# Autodesk Inventor assembly: rotBaseCase
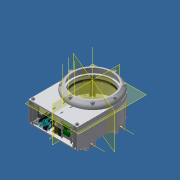
[picture p0: Inventor's stored thumbnail of the model, 180x180]
Saved by Autodesk Inventor 2016 (Build 200138000, 138)
## iProperties
Created: 2016-02-29
Part Number: rotBaseCase
Material: Generisch
Document SubType Name: Assembly
Designer: 4ndreas
Mass: 3728.71 g
Surface Area: 10018.9 cm^2
Volume: 2081.83 cm^3
Density: 1.79108 g/cm^3
Parent: World
Author: 4ndreas
## Documents named in this file (20)
- C:\Users\4ndreas\Documents\github\Mantis-Robot-Arm\MantisRobotArm\Workspace\_assemblys\rotBaseCase.iam
- C:\Users\4ndreas\Documents\github\Mantis-Robot-Arm\MantisRobotArm\Workspace\_metal parts\BasePlate_B.ipt
- C:\Users\4ndreas\Documents\github\Mantis-Robot-Arm\MantisRobotArm\Workspace\_printed parts\BaseBearingMount.ipt
- C:\Users\4ndreas\Documents\github\Mantis-Robot-Arm\MantisRobotArm\Workspace\_assemblys\RotMotor.iam
- C:\Users\4ndreas\Documents\github\Mantis-Robot-Arm\MantisRobotArm\Workspace\_metal parts\Alu_Cover_A.ipt
- C:\Users\4ndreas\Documents\github\Mantis-Robot-Arm\MantisRobotArm\Workspace\_standard Parts\GummiFeet.ipt
- C:\Users\4ndreas\Documents\github\Mantis-Robot-Arm\MantisRobotArm\Libraries\Content Center Files\de-DE\DIN 912\DIN 912 - M5 x 0,8 x 16 x 14.ipt
- C:\Users\4ndreas\Documents\github\Mantis-Robot-Arm\MantisRobotArm\Libraries\Content Center Files\de-DE\DIN 9021\DIN 9021 - 5,3.ipt
- C:\Users\4ndreas\Documents\github\Mantis-Robot-Arm\MantisRobotArm\Workspace\_motors\StepperDriver.ipt
- C:\Users\4ndreas\Documents\github\Mantis-Robot-Arm\MantisRobotArm\Workspace\_metal parts\CAP 0_0_370_03_000   Profil 5  20x20 natur-.ipt
- C:\Users\4ndreas\Documents\github\Mantis-Robot-Arm\MantisRobotArm\Workspace\_metal parts\DriverMount.ipt
- C:\Users\4ndreas\Documents\github\Mantis-Robot-Arm\MantisRobotArm\Libraries\Content Center Files\de-DE\ISO 7380-1\ISO 7380-1 - M3 x 6.ipt
- C:\Users\4ndreas\Documents\github\Mantis-Robot-Arm\MantisRobotArm\Libraries\Content Center Files\de-DE\DIN 912\DIN 912 - M4 x 0,7 x 40 x 20.ipt
- C:\Users\4ndreas\Documents\github\Mantis-Robot-Arm\MantisRobotArm\Libraries\Content Center Files\de-DE\DIN 912\DIN 912 - M4 x 0,7 x 25 x 23,25.ipt
- C:\Users\4ndreas\Documents\github\Mantis-Robot-Arm\MantisRobotArm\Workspace\_metal parts\Distanzhuelse_M3x5mm_.ipt
- C:\Users\4ndreas\Documents\github\Mantis-Robot-Arm\MantisRobotArm\Workspace\_metal parts\Distanzhuelse_M3x20mm_.ipt
- C:\Users\4ndreas\Documents\github\Mantis-Robot-Arm\MantisRobotArm\Workspace\_metal parts\BasePlate_base.ipt
- C:\Users\4ndreas\Documents\github\Mantis-Robot-Arm\MantisRobotArm\Libraries\Content Center Files\arduino due.ipt
- C:\Users\4ndreas\Documents\github\Mantis-Robot-Arm\MantisRobotArm\Workspace\_printed parts\_baseBearingMount.ipt
- C:\Users\4ndreas\Documents\github\Mantis-Robot-Arm\MantisRobotArm\Workspace\_standard Parts\Linearwagen_16_kurz.ipt
## Components (86 placed, 19 different names)
1. BasePlate_base:1 — Passend:2, Passend:11, Passend:12, Passend:13, Passend:14, Passend:15, Passend:16, Passend:17, Passend:18, Passend:19, Passend:20, Passend:21, Passend:22, Passend:34, Fluchtend:8, Passend:36, Passend:37, Passend:40, Passend:41, Passend:42, Passend:119, Passend:163, Passend:172, Passend:173, Fluchtend:42, Passend:183, Passend:184, Tangential:2, Winkel:1, Tangential:3, Passend:187, Passend:188
2. BasePlate_B:1 — Passend:1, Passend:2, Passend:3, Passend:4, Passend:5, Passend:6, Passend:10, Fluchtend:4, Passend:25, Passend:28, Passend:29, Passend:30, Passend:35, Passend:38, Passend:39, Fluchtend:9, Passend:43, Passend:44, Passend:45, Fluchtend:10, Fluchtend:11, Passend:182, Winkel:2
3. BaseBearingMount:1 — Passend:4, Passend:5, Passend:108, Einfügen:1, Einfügen:2, Einfügen:3, Einfügen:4, Einfügen:5, Einfügen:6, Einfügen:7, Einfügen:8
4. RotMotor:1 [sub-assembly] — Passend:6, Passend:9, Passend:1, Passend:182, Passend:190
5. Alu_Cover_A:1 — Passend:9, Passend:10, Fluchtend:4, Tangential:1
6. GummiFeet:1 — Passend:11, Passend:12
7. GummiFeet:2 — Passend:13, Passend:20
8. GummiFeet:3 — Passend:15, Passend:18, Passend:3
9. GummiFeet:4 — Passend:14, Passend:19
10. GummiFeet:5 — Passend:17, Passend:21
11. GummiFeet:6 — Passend:16, Passend:22
12. DIN 912 - ersetzt durch DIN EN ISO 4762 M5 x 16:1 — Passend:23, Passend:24, Passend:25
13. DIN 9021 5,3:1 — Passend:23, Passend:24, Passend:28
14. DIN 912 - ersetzt durch DIN EN ISO 4762 M5 x 16:2 — Passend:29
15. DIN 9021 5,3:2 — Passend:30
16. CAP 0_0_370_03_000   Profil 5  20x20 natur-:1 — Passend:34, Passend:35, Fluchtend:8, Fluchtend:32, Passend:61, Passend:63, Passend:72, Fluchtend:37
17. CAP 0_0_370_03_000   Profil 5  20x20 natur-:2 — Passend:36, Passend:38, Fluchtend:9, Passend:62, Fluchtend:40
18. CAP 0_0_370_03_000   Profil 5  20x20 natur-:3 — Passend:37, Passend:39, Passend:108
19. CAP 0_0_370_03_000   Profil 5  20x20 natur-:4 — Passend:40, Passend:44
20. CAP 0_0_370_03_000   Profil 5  20x20 natur-:5 — Passend:41, Passend:45, Fluchtend:10, Fluchtend:35, Passend:66, Passend:67, Fluchtend:41, Passend:180
21. CAP 0_0_370_03_000   Profil 5  20x20 natur-:6 — Passend:42, Passend:43, Fluchtend:11
22. StepperDriver:6 — Fluchtend:23, Fluchtend:24, Passend:62, Passend:64, Passend:74, Passend:75, Passend:76, Passend:77, Passend:78, Passend:79, Passend:80, Passend:81
23. StepperDriver:8 — Fluchtend:23, Fluchtend:24, Fluchtend:32, Fluchtend:34, Passend:61, Passend:65, Passend:82, Passend:83, Passend:84, Passend:85, Passend:86, Passend:87, Passend:88, Passend:89, Passend:90, Passend:91
24. StepperDriver:10 — Fluchtend:33, Fluchtend:35, Fluchtend:36, Passend:70, Passend:71, Passend:100, Passend:101, Passend:102, Passend:103, Passend:104, Passend:105, Passend:106, Passend:107
25. StepperDriver:11 — Fluchtend:33, Fluchtend:34, Fluchtend:36, Passend:68, Passend:69, Passend:92, Passend:93, Passend:94, Passend:95, Passend:96, Passend:97, Passend:98, Passend:99
26. StepperDriver:12 — Fluchtend:37, Fluchtend:38, Fluchtend:39, Passend:72, Passend:117, Passend:118, Passend:120, Passend:121, Passend:122, Passend:123, Passend:124, Passend:125, Passend:126, Passend:127, Passend:140, Passend:141, Passend:142
27. StepperDriver:13 — Fluchtend:38, Fluchtend:39, Passend:130, Passend:137, Passend:138, Passend:139, Passend:143, Passend:144, Passend:145, Passend:146, Passend:147, Passend:148, Passend:149, Passend:150
28. DriverMount:1 — Fluchtend:40
29. DriverMount:2 — Passend:63, Passend:64, Passend:65
30. DriverMount:3 — Passend:67, Passend:69, Passend:71
31. DriverMount:4 — Passend:66, Passend:68, Passend:70, Fluchtend:41
32. ISO 7380-1 M3 x 6:1 — Passend:74, Passend:75
33. ISO 7380-1 M3 x 6:2 — Passend:76, Passend:77
34. ISO 7380-1 M3 x 6:3 — Passend:78, Passend:79
35. ISO 7380-1 M3 x 6:4 — Passend:80, Passend:81
36. ISO 7380-1 M3 x 6:5 — Passend:82, Passend:83
37. ISO 7380-1 M3 x 6:6 — Passend:84, Passend:85
38. ISO 7380-1 M3 x 6:7 — Passend:86, Passend:87
39. ISO 7380-1 M3 x 6:8 — Passend:88, Passend:89
40. ISO 7380-1 M3 x 6:9 — Passend:90, Passend:91
41. ISO 7380-1 M3 x 6:10 — Passend:92, Passend:93
42. ISO 7380-1 M3 x 6:11 — Passend:94, Passend:95
43. ISO 7380-1 M3 x 6:12 — Passend:96, Passend:97
44. ISO 7380-1 M3 x 6:13 — Passend:98, Passend:99
45. ISO 7380-1 M3 x 6:14 — Passend:100, Passend:101
46. ISO 7380-1 M3 x 6:15 — Passend:102, Passend:103
47. ISO 7380-1 M3 x 6:16 — Passend:104, Passend:105
48. ISO 7380-1 M3 x 6:17 — Passend:106, Passend:107
49. DIN 912 - ersetzt durch DIN EN ISO 4762 M4 x 40:1 — Einfügen:1
50. DIN 912 - ersetzt durch DIN EN ISO 4762 M4 x 25:2 — Einfügen:2
51. DIN 912 - ersetzt durch DIN EN ISO 4762 M4 x 25:5 — Einfügen:3
52. DIN 912 - ersetzt durch DIN EN ISO 4762 M4 x 25:6 — Einfügen:4
53. DIN 912 - ersetzt durch DIN EN ISO 4762 M4 x 25:4 — Einfügen:5
54. DIN 912 - ersetzt durch DIN EN ISO 4762 M4 x 25:3 — Einfügen:6
55. DIN 912 - ersetzt durch DIN EN ISO 4762 M4 x 40:7 — Einfügen:7
56. DIN 912 - ersetzt durch DIN EN ISO 4762 M4 x 25:1 — Einfügen:8
57. Distanzhuelse_M3x5mm_:1 — Passend:163, Passend:164, Passend:166
58. Distanzhuelse_M3x20mm_:1 — Passend:117, Passend:118, Passend:119
59. Distanzhuelse_M3x5mm_:3 — Passend:174, Passend:177
60. Distanzhuelse_M3x5mm_:4 — Passend:175, Passend:176
61. Distanzhuelse_M3x5mm_:5 — Passend:178, Passend:179
62. Distanzhuelse_M3x20mm_:2 — Passend:122, Passend:123
63. Distanzhuelse_M3x20mm_:3 — Passend:121, Passend:124
64. Distanzhuelse_M3x20mm_:4 — Passend:120, Passend:125
65. Distanzhuelse_M3x20mm_:5 — Passend:126, Passend:127, Passend:128, Passend:129
66. Distanzhuelse_M3x20mm_:6 — Passend:128, Passend:129, Passend:130
67. Distanzhuelse_M3x20mm_:7 — Passend:131, Passend:134, Passend:142
68. Distanzhuelse_M3x20mm_:8 — Passend:132, Passend:135, Passend:140
69. Distanzhuelse_M3x20mm_:9 — Passend:131, Passend:134, Passend:137
70. Distanzhuelse_M3x20mm_:10 — Passend:132, Passend:135, Passend:138
71. Distanzhuelse_M3x20mm_:11 — Passend:133, Passend:136, Passend:141
72. Distanzhuelse_M3x20mm_:12 — Passend:133, Passend:136, Passend:139
73. ISO 7380-1 M3 x 6:18 — Passend:143, Passend:144
74. ISO 7380-1 M3 x 6:19 — Passend:145, Passend:146
75. ISO 7380-1 M3 x 6:20 — Passend:147, Passend:148
76. ISO 7380-1 M3 x 6:21 — Passend:149, Passend:150
77. ISO 7380-1 M3 x 6:22 — Passend:165, Passend:166
78. ISO 7380-1 M3 x 6:25 — Passend:168, Passend:169, Passend:174
79. ISO 7380-1 M3 x 6:26 — Passend:170, Passend:171, Passend:175
80. ISO 7380-1 M3 x 6:27 — Passend:167, Passend:178
81. arduino due:1 — Passend:164, Passend:165, Passend:167, Passend:168, Passend:169, Passend:170, Passend:171, Passend:176, Passend:177, Fluchtend:42, Passend:179, Passend:180
82. _baseBearingMount:1 — Passend:172, Passend:173, Passend:191
83. Linearwagen_16_kurz:1 — Passend:183, Passend:185, Tangential:1, Tangential:2, Winkel:1, Fluchtend:43
84. Linearwagen_16_kurz:2 — Passend:184, Passend:185, Tangential:3, Fluchtend:44, Passend:189
85. Linearwagen_16_kurz:3 — Passend:186, Passend:187, Fluchtend:43
86. Linearwagen_16_kurz:4 — Passend:186, Passend:188, Fluchtend:44, Passend:189
## Relationships (185: Mate 149, Flush 23, Insert 8, Tangent 3, Angle 2)
- Passend:1 [Mate]: BasePlate_B:1 ↔ RotMotor:1
- Passend:2 [Mate] (85 mm): BasePlate_base:1 ↔ BasePlate_B:1
- Passend:3 [Mate]: BasePlate_B:1 ↔ GummiFeet:3
- [Flush]: BasePlate_base:1
- [Flush]: BasePlate_base:1
- [Flush]: BasePlate_base:1
- Passend:4 [Mate]: BasePlate_B:1 ↔ BaseBearingMount:1
- Passend:5 [Mate]: BasePlate_B:1 ↔ BaseBearingMount:1
- Passend:6 [Mate]: BasePlate_B:1 ↔ RotMotor:1
- Passend:9 [Mate]: RotMotor:1 ↔ Alu_Cover_A:1
- Passend:10 [Mate]: BasePlate_B:1 ↔ Alu_Cover_A:1
- Fluchtend:4 [Flush]: BasePlate_B:1 ↔ Alu_Cover_A:1
- Passend:11 [Mate]: BasePlate_base:1 ↔ GummiFeet:1
- Passend:12 [Mate]: BasePlate_base:1 ↔ GummiFeet:1
- Passend:13 [Mate]: BasePlate_base:1 ↔ GummiFeet:2
- Passend:14 [Mate]: BasePlate_base:1 ↔ GummiFeet:4
- Passend:15 [Mate]: BasePlate_base:1 ↔ GummiFeet:3
- Passend:16 [Mate]: BasePlate_base:1 ↔ GummiFeet:6
- Passend:17 [Mate]: BasePlate_base:1 ↔ GummiFeet:5
- Passend:18 [Mate]: BasePlate_base:1 ↔ GummiFeet:3
- Passend:19 [Mate]: BasePlate_base:1 ↔ GummiFeet:4
- Passend:20 [Mate]: BasePlate_base:1 ↔ GummiFeet:2
- Passend:21 [Mate]: BasePlate_base:1 ↔ GummiFeet:5
- Passend:22 [Mate]: BasePlate_base:1 ↔ GummiFeet:6
- Passend:23 [Mate]: DIN 912 - ersetzt durch DIN EN ISO 4762 M5 x 16:1 ↔ DIN 9021 5,3:1
- Passend:24 [Mate]: DIN 912 - ersetzt durch DIN EN ISO 4762 M5 x 16:1 ↔ DIN 9021 5,3:1
- Passend:25 [Mate]: BasePlate_B:1 ↔ DIN 912 - ersetzt durch DIN EN ISO 4762 M5 x 16:1
- [Mate]: DIN 912 - ersetzt durch DIN EN ISO 4762 M5 x 16:2 ↔ DIN 9021 5,3:2
- [Mate]: DIN 912 - ersetzt durch DIN EN ISO 4762 M5 x 16:2 ↔ DIN 9021 5,3:2
- Passend:28 [Mate]: BasePlate_B:1 ↔ DIN 9021 5,3:1
- Passend:29 [Mate]: BasePlate_B:1 ↔ DIN 912 - ersetzt durch DIN EN ISO 4762 M5 x 16:2
- Passend:30 [Mate]: BasePlate_B:1 ↔ DIN 9021 5,3:2
- Passend:34 [Mate]: BasePlate_base:1 ↔ CAP 0_0_370_03_000   Profil 5  20x20 natur-:1
- Passend:35 [Mate]: BasePlate_B:1 ↔ CAP 0_0_370_03_000   Profil 5  20x20 natur-:1
- Fluchtend:8 [Flush]: BasePlate_base:1 ↔ CAP 0_0_370_03_000   Profil 5  20x20 natur-:1
- Passend:36 [Mate]: BasePlate_base:1 ↔ CAP 0_0_370_03_000   Profil 5  20x20 natur-:2
- Passend:37 [Mate]: BasePlate_base:1 ↔ CAP 0_0_370_03_000   Profil 5  20x20 natur-:3
- Passend:38 [Mate]: BasePlate_B:1 ↔ CAP 0_0_370_03_000   Profil 5  20x20 natur-:2
- Passend:39 [Mate]: BasePlate_B:1 ↔ CAP 0_0_370_03_000   Profil 5  20x20 natur-:3
- Fluchtend:9 [Flush]: BasePlate_B:1 ↔ CAP 0_0_370_03_000   Profil 5  20x20 natur-:2
- Passend:40 [Mate]: BasePlate_base:1 ↔ CAP 0_0_370_03_000   Profil 5  20x20 natur-:4
- Passend:41 [Mate]: BasePlate_base:1 ↔ CAP 0_0_370_03_000   Profil 5  20x20 natur-:5
- Passend:42 [Mate]: BasePlate_base:1 ↔ CAP 0_0_370_03_000   Profil 5  20x20 natur-:6
- Passend:43 [Mate]: BasePlate_B:1 ↔ CAP 0_0_370_03_000   Profil 5  20x20 natur-:6
- Passend:44 [Mate]: BasePlate_B:1 ↔ CAP 0_0_370_03_000   Profil 5  20x20 natur-:4
- Passend:45 [Mate]: BasePlate_B:1 ↔ CAP 0_0_370_03_000   Profil 5  20x20 natur-:5
- Fluchtend:10 [Flush]: BasePlate_B:1 ↔ CAP 0_0_370_03_000   Profil 5  20x20 natur-:5
- Fluchtend:11 [Flush]: BasePlate_B:1 ↔ CAP 0_0_370_03_000   Profil 5  20x20 natur-:6
- Fluchtend:23 [Flush]: StepperDriver:6 ↔ StepperDriver:8
- Fluchtend:24 [Flush]: StepperDriver:6 ↔ StepperDriver:8
- Fluchtend:32 [Flush]: CAP 0_0_370_03_000   Profil 5  20x20 natur-:1 ↔ StepperDriver:8
- Fluchtend:33 [Flush]: StepperDriver:10 ↔ StepperDriver:11
- Fluchtend:34 [Flush]: StepperDriver:8 ↔ StepperDriver:11
- Fluchtend:35 [Flush]: CAP 0_0_370_03_000   Profil 5  20x20 natur-:5 ↔ StepperDriver:10
- Fluchtend:36 [Flush]: StepperDriver:10 ↔ StepperDriver:11
- Fluchtend:37 [Flush] (10 mm): CAP 0_0_370_03_000   Profil 5  20x20 natur-:1 ↔ StepperDriver:12
- Fluchtend:38 [Flush]: StepperDriver:12 ↔ StepperDriver:13
- Fluchtend:39 [Flush]: StepperDriver:12 ↔ StepperDriver:13
- Passend:61 [Mate] (2 mm): CAP 0_0_370_03_000   Profil 5  20x20 natur-:1 ↔ StepperDriver:8
- Passend:62 [Mate] (2 mm): CAP 0_0_370_03_000   Profil 5  20x20 natur-:2 ↔ StepperDriver:6
- Fluchtend:40 [Flush]: CAP 0_0_370_03_000   Profil 5  20x20 natur-:2 ↔ DriverMount:1
- Passend:63 [Mate]: CAP 0_0_370_03_000   Profil 5  20x20 natur-:1 ↔ DriverMount:2
- Passend:64 [Mate]: StepperDriver:6 ↔ DriverMount:2
- Passend:65 [Mate]: StepperDriver:8 ↔ DriverMount:2
- Passend:66 [Mate]: CAP 0_0_370_03_000   Profil 5  20x20 natur-:5 ↔ DriverMount:4
- Passend:67 [Mate]: CAP 0_0_370_03_000   Profil 5  20x20 natur-:5 ↔ DriverMount:3
- Passend:68 [Mate]: StepperDriver:11 ↔ DriverMount:4
- Passend:69 [Mate]: StepperDriver:11 ↔ DriverMount:3
- Passend:70 [Mate]: StepperDriver:10 ↔ DriverMount:4
- Fluchtend:41 [Flush]: CAP 0_0_370_03_000   Profil 5  20x20 natur-:5 ↔ DriverMount:4
- Passend:71 [Mate]: StepperDriver:10 ↔ DriverMount:3
- Passend:72 [Mate] (16 mm): CAP 0_0_370_03_000   Profil 5  20x20 natur-:1 ↔ StepperDriver:12
- Passend:74 [Mate]: StepperDriver:6 ↔ ISO 7380-1 M3 x 6:1
- Passend:75 [Mate]: StepperDriver:6 ↔ ISO 7380-1 M3 x 6:1
- Passend:76 [Mate]: StepperDriver:6 ↔ ISO 7380-1 M3 x 6:2
- Passend:77 [Mate]: StepperDriver:6 ↔ ISO 7380-1 M3 x 6:2
- Passend:78 [Mate]: StepperDriver:6 ↔ ISO 7380-1 M3 x 6:3
- Passend:79 [Mate]: StepperDriver:6 ↔ ISO 7380-1 M3 x 6:3
- Passend:80 [Mate]: StepperDriver:6 ↔ ISO 7380-1 M3 x 6:4
- Passend:81 [Mate]: StepperDriver:6 ↔ ISO 7380-1 M3 x 6:4
- Passend:82 [Mate]: StepperDriver:8 ↔ ISO 7380-1 M3 x 6:5
- Passend:83 [Mate]: StepperDriver:8 ↔ ISO 7380-1 M3 x 6:5
- Passend:84 [Mate]: StepperDriver:8 ↔ ISO 7380-1 M3 x 6:6
- Passend:85 [Mate]: StepperDriver:8 ↔ ISO 7380-1 M3 x 6:6
- Passend:86 [Mate]: StepperDriver:8 ↔ ISO 7380-1 M3 x 6:7
- Passend:87 [Mate]: StepperDriver:8 ↔ ISO 7380-1 M3 x 6:7
- Passend:88 [Mate]: StepperDriver:8 ↔ ISO 7380-1 M3 x 6:8
- Passend:89 [Mate]: StepperDriver:8 ↔ ISO 7380-1 M3 x 6:8
- Passend:90 [Mate]: StepperDriver:8 ↔ ISO 7380-1 M3 x 6:9
- Passend:91 [Mate]: StepperDriver:8 ↔ ISO 7380-1 M3 x 6:9
- Passend:92 [Mate]: StepperDriver:11 ↔ ISO 7380-1 M3 x 6:10
- Passend:93 [Mate]: StepperDriver:11 ↔ ISO 7380-1 M3 x 6:10
- Passend:94 [Mate]: StepperDriver:11 ↔ ISO 7380-1 M3 x 6:11
- Passend:95 [Mate]: StepperDriver:11 ↔ ISO 7380-1 M3 x 6:11
- Passend:96 [Mate]: StepperDriver:11 ↔ ISO 7380-1 M3 x 6:12
- Passend:97 [Mate]: StepperDriver:11 ↔ ISO 7380-1 M3 x 6:12
- Passend:98 [Mate]: StepperDriver:11 ↔ ISO 7380-1 M3 x 6:13
- Passend:99 [Mate]: StepperDriver:11 ↔ ISO 7380-1 M3 x 6:13
- Passend:100 [Mate]: StepperDriver:10 ↔ ISO 7380-1 M3 x 6:14
- Passend:101 [Mate]: StepperDriver:10 ↔ ISO 7380-1 M3 x 6:14
- Passend:102 [Mate]: StepperDriver:10 ↔ ISO 7380-1 M3 x 6:15
- Passend:103 [Mate]: StepperDriver:10 ↔ ISO 7380-1 M3 x 6:15
- Passend:104 [Mate]: StepperDriver:10 ↔ ISO 7380-1 M3 x 6:16
- Passend:105 [Mate]: StepperDriver:10 ↔ ISO 7380-1 M3 x 6:16
- Passend:106 [Mate]: StepperDriver:10 ↔ ISO 7380-1 M3 x 6:17
- Passend:107 [Mate]: StepperDriver:10 ↔ ISO 7380-1 M3 x 6:17
- Passend:108 [Mate]: BaseBearingMount:1 ↔ CAP 0_0_370_03_000   Profil 5  20x20 natur-:3
- Einfügen:1 [Insert]: BaseBearingMount:1 ↔ DIN 912 - ersetzt durch DIN EN ISO 4762 M4 x 40:1
- Einfügen:2 [Insert]: BaseBearingMount:1 ↔ DIN 912 - ersetzt durch DIN EN ISO 4762 M4 x 25:2
- Einfügen:3 [Insert]: BaseBearingMount:1 ↔ DIN 912 - ersetzt durch DIN EN ISO 4762 M4 x 25:5
- Einfügen:4 [Insert]: BaseBearingMount:1 ↔ DIN 912 - ersetzt durch DIN EN ISO 4762 M4 x 25:6
- Einfügen:5 [Insert]: BaseBearingMount:1 ↔ DIN 912 - ersetzt durch DIN EN ISO 4762 M4 x 25:4
- Einfügen:6 [Insert]: BaseBearingMount:1 ↔ DIN 912 - ersetzt durch DIN EN ISO 4762 M4 x 25:3
- Einfügen:7 [Insert]: BaseBearingMount:1 ↔ DIN 912 - ersetzt durch DIN EN ISO 4762 M4 x 40:7
- Einfügen:8 [Insert]: BaseBearingMount:1 ↔ DIN 912 - ersetzt durch DIN EN ISO 4762 M4 x 25:1
- Passend:117 [Mate]: StepperDriver:12 ↔ Distanzhuelse_M3x20mm_:1
- Passend:118 [Mate]: StepperDriver:12 ↔ Distanzhuelse_M3x20mm_:1
- Passend:119 [Mate]: BasePlate_base:1 ↔ Distanzhuelse_M3x20mm_:1
- Passend:120 [Mate]: StepperDriver:12 ↔ Distanzhuelse_M3x20mm_:4
- Passend:121 [Mate]: StepperDriver:12 ↔ Distanzhuelse_M3x20mm_:3
- Passend:122 [Mate]: StepperDriver:12 ↔ Distanzhuelse_M3x20mm_:2
- Passend:123 [Mate]: StepperDriver:12 ↔ Distanzhuelse_M3x20mm_:2
- Passend:124 [Mate]: StepperDriver:12 ↔ Distanzhuelse_M3x20mm_:3
- Passend:125 [Mate]: StepperDriver:12 ↔ Distanzhuelse_M3x20mm_:4
- Passend:126 [Mate]: StepperDriver:12 ↔ Distanzhuelse_M3x20mm_:5
- Passend:127 [Mate]: StepperDriver:12 ↔ Distanzhuelse_M3x20mm_:5
- Passend:128 [Mate]: Distanzhuelse_M3x20mm_:5 ↔ Distanzhuelse_M3x20mm_:6
- Passend:129 [Mate]: Distanzhuelse_M3x20mm_:5 ↔ Distanzhuelse_M3x20mm_:6
- Passend:130 [Mate]: StepperDriver:13 ↔ Distanzhuelse_M3x20mm_:6
- Passend:131 [Mate]: Distanzhuelse_M3x20mm_:7 ↔ Distanzhuelse_M3x20mm_:9
- Passend:132 [Mate]: Distanzhuelse_M3x20mm_:8 ↔ Distanzhuelse_M3x20mm_:10
- Passend:133 [Mate]: Distanzhuelse_M3x20mm_:11 ↔ Distanzhuelse_M3x20mm_:12
- Passend:134 [Mate]: Distanzhuelse_M3x20mm_:7 ↔ Distanzhuelse_M3x20mm_:9
- Passend:135 [Mate]: Distanzhuelse_M3x20mm_:8 ↔ Distanzhuelse_M3x20mm_:10
- Passend:136 [Mate]: Distanzhuelse_M3x20mm_:11 ↔ Distanzhuelse_M3x20mm_:12
- Passend:137 [Mate]: StepperDriver:13 ↔ Distanzhuelse_M3x20mm_:9
- Passend:138 [Mate]: StepperDriver:13 ↔ Distanzhuelse_M3x20mm_:10
- Passend:139 [Mate]: StepperDriver:13 ↔ Distanzhuelse_M3x20mm_:12
- Passend:140 [Mate]: StepperDriver:12 ↔ Distanzhuelse_M3x20mm_:8
- Passend:141 [Mate]: StepperDriver:12 ↔ Distanzhuelse_M3x20mm_:11
- Passend:142 [Mate]: StepperDriver:12 ↔ Distanzhuelse_M3x20mm_:7
- Passend:143 [Mate]: StepperDriver:13 ↔ ISO 7380-1 M3 x 6:18
- Passend:144 [Mate]: StepperDriver:13 ↔ ISO 7380-1 M3 x 6:18
- Passend:145 [Mate]: StepperDriver:13 ↔ ISO 7380-1 M3 x 6:19
- Passend:146 [Mate]: StepperDriver:13 ↔ ISO 7380-1 M3 x 6:19
- Passend:147 [Mate]: StepperDriver:13 ↔ ISO 7380-1 M3 x 6:20
- Passend:148 [Mate]: StepperDriver:13 ↔ ISO 7380-1 M3 x 6:20
- Passend:149 [Mate]: StepperDriver:13 ↔ ISO 7380-1 M3 x 6:21
- Passend:150 [Mate]: StepperDriver:13 ↔ ISO 7380-1 M3 x 6:21
- Passend:163 [Mate]: BasePlate_base:1 ↔ Distanzhuelse_M3x5mm_:1
- Passend:164 [Mate]: Distanzhuelse_M3x5mm_:1 ↔ arduino due:1
- Passend:165 [Mate]: ISO 7380-1 M3 x 6:22 ↔ arduino due:1
- Passend:166 [Mate]: Distanzhuelse_M3x5mm_:1 ↔ ISO 7380-1 M3 x 6:22
- Passend:167 [Mate]: ISO 7380-1 M3 x 6:27 ↔ arduino due:1
- Passend:168 [Mate]: ISO 7380-1 M3 x 6:25 ↔ arduino due:1
- Passend:169 [Mate]: ISO 7380-1 M3 x 6:25 ↔ arduino due:1
- Passend:170 [Mate]: ISO 7380-1 M3 x 6:26 ↔ arduino due:1
- Passend:171 [Mate]: ISO 7380-1 M3 x 6:26 ↔ arduino due:1
- Passend:172 [Mate]: BasePlate_base:1 ↔ _baseBearingMount:1
- Passend:173 [Mate]: BasePlate_base:1 ↔ _baseBearingMount:1
- Passend:174 [Mate]: Distanzhuelse_M3x5mm_:3 ↔ ISO 7380-1 M3 x 6:25
- Passend:175 [Mate]: Distanzhuelse_M3x5mm_:4 ↔ ISO 7380-1 M3 x 6:26
- Passend:176 [Mate]: Distanzhuelse_M3x5mm_:4 ↔ arduino due:1
- Passend:177 [Mate]: Distanzhuelse_M3x5mm_:3 ↔ arduino due:1
- Fluchtend:42 [Flush]: BasePlate_base:1 ↔ arduino due:1
- Passend:178 [Mate]: Distanzhuelse_M3x5mm_:5 ↔ ISO 7380-1 M3 x 6:27
- Passend:179 [Mate]: Distanzhuelse_M3x5mm_:5 ↔ arduino due:1
- Passend:180 [Mate] (8 mm): CAP 0_0_370_03_000   Profil 5  20x20 natur-:5 ↔ arduino due:1
- Passend:182 [Mate]: BasePlate_B:1 ↔ RotMotor:1
- Passend:183 [Mate]: BasePlate_base:1 ↔ Linearwagen_16_kurz:1
- Passend:184 [Mate]: BasePlate_base:1 ↔ Linearwagen_16_kurz:2
- Passend:185 [Mate]: Linearwagen_16_kurz:1 ↔ Linearwagen_16_kurz:2
- Tangential:1: Alu_Cover_A:1 ↔ Linearwagen_16_kurz:1
- Tangential:2: BasePlate_base:1 ↔ Linearwagen_16_kurz:1
- Winkel:1 [Angle] (0 deg): BasePlate_base:1 ↔ Linearwagen_16_kurz:1
- Tangential:3: BasePlate_base:1 ↔ Linearwagen_16_kurz:2
- Passend:186 [Mate]: Linearwagen_16_kurz:3 ↔ Linearwagen_16_kurz:4
- Passend:187 [Mate]: BasePlate_base:1 ↔ Linearwagen_16_kurz:3
- Passend:188 [Mate]: BasePlate_base:1 ↔ Linearwagen_16_kurz:4
- Fluchtend:43 [Flush]: Linearwagen_16_kurz:1 ↔ Linearwagen_16_kurz:3
- Fluchtend:44 [Flush]: Linearwagen_16_kurz:2 ↔ Linearwagen_16_kurz:4
- Passend:189 [Mate] (135 mm): Linearwagen_16_kurz:2 ↔ Linearwagen_16_kurz:4
- Passend:190 [Mate]: RotMotor:1
- Winkel:2 [Angle] (22.5 deg): BasePlate_B:1
- Passend:191 [Mate]: _baseBearingMount:1
## Named parameters: d30_d27 = 0 mm, d31_d28 = 0 mm
